# Autodesk Inventor assembly: smartboard1
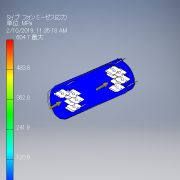
[picture p0: Inventor's stored thumbnail of the model, 180x180]
Saved by Autodesk Inventor 2019 (Build 230136000, 136)
## iProperties
Created: 2019-02-09
Part Number: smartboard1
Material: 一般
Document SubType Name: Assembly
Designer: drago
Author: drago
## Documents named in this file (15)
- C:\Users\drago\Documents\SFP\sfp_smartboard\smartboard1.iam
- C:\Users\drago\Documents\SFP\sfp_smartboard\sfp_smartboard_lower_deck.ipt
- C:\Users\drago\Documents\SFP\sfp_smartboard\track_data\Truck.iam
- C:\Users\drago\Documents\Inventor\Content Center Files\R2019\ja-JP\DIN 7991(2)\DIN 7991 - M5x20.ipt
- C:\Users\drago\Documents\Inventor\Content Center Files\R2019\ja-JP\AS 1112 (2)\AS 1112 - M5  Type 5.ipt
- C:\Users\drago\Documents\SFP\sfp_smartboard\sc601_load_cell.ipt
- C:\Users\drago\Documents\Inventor\Content Center Files\R2019\ja-JP\AS 1112 (2)\AS 1112 - M6  Type 5.ipt
- C:\Users\drago\Documents\Inventor\Content Center Files\R2019\ja-JP\AS 1427(04)\AS 1427 - M6 x 50(5) I.ipt
- C:\Users\drago\Documents\SFP\sfp_smartboard\sfp_smartboard_upper_deck.ipt
- C:\Users\drago\Documents\SFP\sfp_smartboard\smartboard1\AIP\FEA\cs536vov4.fins
- C:\Users\drago\Documents\SFP\sfp_smartboard\smartboard1\AIP\FEA\cs536vow0.fsat
- C:\Users\drago\Documents\SFP\sfp_smartboard\smartboard1\AIP\FEA\cs536vow0.ftes
- C:\Users\drago\Documents\SFP\sfp_smartboard\smartboard1\AIP\FEA\cs536vow0.fwiz
- C:\Users\drago\Documents\SFP\sfp_smartboard\smartboard1\AIP\FEA\cs536vp6o.fmsh
- C:\Users\drago\Documents\SFP\sfp_smartboard\smartboard1\AIP\FEA\cs536vp6p.fres
## Components (54 placed, 8 different names)
1. sfp_smartboard_lower_deck:1 — 挿入:2, 挿入:3, 挿入:4, 挿入:5, 挿入:6, 挿入:7, 挿入:8, 挿入:9, 挿入:10, 挿入:11, 挿入:12, 挿入:13, メイト:1, メイト:2, 挿入:22, 挿入:24, メイト:6, メイト:7, 挿入:27, 挿入:29
2. Truck:1 [sub-assembly] — 挿入:9, 挿入:10, 挿入:18, 挿入:19, 挿入:20, 挿入:21
3. Truck:2 [sub-assembly] — 挿入:11, 挿入:13, 挿入:14, 挿入:15, 挿入:16, 挿入:17
4. DIN 7991 M5x20:1 — 挿入:12
5. DIN 7991 M5x20:3 — 挿入:3
6. DIN 7991 M5x20:4 — 挿入:2
7. DIN 7991 M5x20:5 — 挿入:4
8. DIN 7991 M5x20:6 — 挿入:7
9. DIN 7991 M5x20:7 — 挿入:8
10. DIN 7991 M5x20:8 — 挿入:6
11. DIN 7991 M5x20:9 — 挿入:5
12. AS 1112 (2) - Metric M5  Type 5:1 — 挿入:14
13. AS 1112 (2) - Metric M5  Type 5:2 — 挿入:15
14. AS 1112 (2) - Metric M5  Type 5:3 — 挿入:16
15. AS 1112 (2) - Metric M5  Type 5:4 — 挿入:17
16. AS 1112 (2) - Metric M5  Type 5:5 — 挿入:18
17. AS 1112 (2) - Metric M5  Type 5:6 — 挿入:19
18. AS 1112 (2) - Metric M5  Type 5:7 — 挿入:20
19. AS 1112 (2) - Metric M5  Type 5:8 — 挿入:21
20. sc601_load_cell:1 — 挿入:31, 挿入:32, 挿入:33, 挿入:34, 挿入:47, 挿入:51, 挿入:52
21. sc601_load_cell:2 — 挿入:26, メイト:3, メイト:4, メイト:5, 挿入:48, 挿入:49, 挿入:50
22. AS 1112 (2) - Metric M6  Type 5:1 — 挿入:43, 挿入:45
23. AS 1112 (2) - Metric M6  Type 5:2 — 挿入:45, 挿入:47
24. AS 1112 (2) - Metric M6  Type 5:3 — 挿入:42, 挿入:48
25. AS 1112 (2) - Metric M6  Type 5:4 — 挿入:24, 挿入:25
26. AS 1112 (2) - Metric M6  Type 5:5 — 挿入:23, 挿入:26
27. AS 1112 (2) - Metric M6  Type 5:6 — 挿入:22, 挿入:23
28. AS 1112 (2) - Metric M6  Type 5:7 — 挿入:41
29. AS 1112 (2) - Metric M6  Type 5:8 — 挿入:25, メイト:3
30. AS 1112 (2) - Metric M6  Type 5:9 — メイト:4
31. AS 1112 (2) - Metric M6  Type 5:10 — 挿入:44, 挿入:46
32. AS 1112 (2) - Metric M6  Type 5:11 — メイト:5
33. AS 1112 (2) - Metric M6  Type 5:12 — 挿入:40, 挿入:42
34. AS 1112 (2) - Metric M6  Type 5:13 — 挿入:39, 挿入:41
35. AS 1112 (2) - Metric M6  Type 5:14 — 挿入:27, 挿入:28
36. AS 1112 (2) - Metric M6  Type 5:15 — 挿入:51
37. AS 1112 (2) - Metric M6  Type 5:16 — 挿入:52
38. AS 1112 (2) - Metric M6  Type 5:17 — 挿入:28, 挿入:32
39. AS 1112 (2) - Metric M6  Type 5:18 — 挿入:29, 挿入:30
40. AS 1112 (2) - Metric M6  Type 5:19 — 挿入:50
41. AS 1112 (2) - Metric M6  Type 5:20 — 挿入:46
42. AS 1112 (2) - Metric M6  Type 5:21 — 挿入:33
43. AS 1112 (2) - Metric M6  Type 5:22 — 挿入:34
44. AS 1112 (2) - Metric M6  Type 5:23 — 挿入:49
45. AS 1112 (2) - Metric M6  Type 5:24 — 挿入:30, 挿入:31
46. AS 1427 H - Metric M6 x 50:1 — メイト:1
47. AS 1427 H - Metric M6 x 50:2 — メイト:2
48. AS 1427 H - Metric M6 x 50:7 — メイト:7
49. AS 1427 H - Metric M6 x 50:8 — メイト:6
50. AS 1427 H - Metric M6 x 50:9 — 挿入:36
51. AS 1427 H - Metric M6 x 50:10 — 挿入:37
52. AS 1427 H - Metric M6 x 50:11 — 挿入:38
53. AS 1427 H - Metric M6 x 50:12 — 挿入:35
54. sfp_smartboard_upper_deck:1 — 挿入:35, 挿入:36, 挿入:37, 挿入:38, 挿入:39, 挿入:40, 挿入:43, 挿入:44
## Relationships (58: Insert 51, Mate 7)
- 挿入:2 [Insert]: sfp_smartboard_lower_deck:1 ↔ DIN 7991 M5x20:4
- 挿入:3 [Insert]: sfp_smartboard_lower_deck:1 ↔ DIN 7991 M5x20:3
- 挿入:4 [Insert]: sfp_smartboard_lower_deck:1 ↔ DIN 7991 M5x20:5
- 挿入:5 [Insert]: sfp_smartboard_lower_deck:1 ↔ DIN 7991 M5x20:9
- 挿入:6 [Insert]: sfp_smartboard_lower_deck:1 ↔ DIN 7991 M5x20:8
- 挿入:7 [Insert]: sfp_smartboard_lower_deck:1 ↔ DIN 7991 M5x20:6
- 挿入:8 [Insert]: sfp_smartboard_lower_deck:1 ↔ DIN 7991 M5x20:7
- 挿入:9 [Insert]: sfp_smartboard_lower_deck:1 ↔ Truck:1
- 挿入:10 [Insert]: sfp_smartboard_lower_deck:1 ↔ Truck:1
- 挿入:11 [Insert]: sfp_smartboard_lower_deck:1 ↔ Truck:2
- 挿入:12 [Insert]: sfp_smartboard_lower_deck:1 ↔ DIN 7991 M5x20:1
- 挿入:13 [Insert]: sfp_smartboard_lower_deck:1 ↔ Truck:2
- 挿入:14 [Insert]: Truck:2 ↔ AS 1112 (2) - Metric M5  Type 5:1
- 挿入:15 [Insert]: Truck:2 ↔ AS 1112 (2) - Metric M5  Type 5:2
- 挿入:16 [Insert]: Truck:2 ↔ AS 1112 (2) - Metric M5  Type 5:3
- 挿入:17 [Insert]: Truck:2 ↔ AS 1112 (2) - Metric M5  Type 5:4
- 挿入:18 [Insert]: Truck:1 ↔ AS 1112 (2) - Metric M5  Type 5:5
- 挿入:19 [Insert]: Truck:1 ↔ AS 1112 (2) - Metric M5  Type 5:6
- 挿入:20 [Insert]: Truck:1 ↔ AS 1112 (2) - Metric M5  Type 5:7
- 挿入:21 [Insert]: Truck:1 ↔ AS 1112 (2) - Metric M5  Type 5:8
- メイト:1 [Mate]: sfp_smartboard_lower_deck:1 ↔ AS 1427 H - Metric M6 x 50:1
- メイト:2 [Mate]: sfp_smartboard_lower_deck:1 ↔ AS 1427 H - Metric M6 x 50:2
- 挿入:22 [Insert]: sfp_smartboard_lower_deck:1 ↔ AS 1112 (2) - Metric M6  Type 5:6
- 挿入:23 [Insert]: AS 1112 (2) - Metric M6  Type 5:5 ↔ AS 1112 (2) - Metric M6  Type 5:6
- 挿入:24 [Insert]: sfp_smartboard_lower_deck:1 ↔ AS 1112 (2) - Metric M6  Type 5:4
- 挿入:25 [Insert]: AS 1112 (2) - Metric M6  Type 5:4 ↔ AS 1112 (2) - Metric M6  Type 5:8
- 挿入:26 [Insert]: sc601_load_cell:2 ↔ AS 1112 (2) - Metric M6  Type 5:5
- メイト:3 [Mate]: sc601_load_cell:2 ↔ AS 1112 (2) - Metric M6  Type 5:8
- メイト:4 [Mate]: sc601_load_cell:2 ↔ AS 1112 (2) - Metric M6  Type 5:9
- メイト:5 [Mate]: sc601_load_cell:2 ↔ AS 1112 (2) - Metric M6  Type 5:11
- メイト:6 [Mate]: sfp_smartboard_lower_deck:1 ↔ AS 1427 H - Metric M6 x 50:8
- メイト:7 [Mate]: sfp_smartboard_lower_deck:1 ↔ AS 1427 H - Metric M6 x 50:7
- 挿入:27 [Insert]: sfp_smartboard_lower_deck:1 ↔ AS 1112 (2) - Metric M6  Type 5:14
- 挿入:28 [Insert]: AS 1112 (2) - Metric M6  Type 5:14 ↔ AS 1112 (2) - Metric M6  Type 5:17
- 挿入:29 [Insert]: sfp_smartboard_lower_deck:1 ↔ AS 1112 (2) - Metric M6  Type 5:18
- 挿入:30 [Insert]: AS 1112 (2) - Metric M6  Type 5:18 ↔ AS 1112 (2) - Metric M6  Type 5:24
- 挿入:31 [Insert]: sc601_load_cell:1 ↔ AS 1112 (2) - Metric M6  Type 5:24
- 挿入:32 [Insert]: sc601_load_cell:1 ↔ AS 1112 (2) - Metric M6  Type 5:17
- 挿入:33 [Insert]: sc601_load_cell:1 ↔ AS 1112 (2) - Metric M6  Type 5:21
- 挿入:34 [Insert]: sc601_load_cell:1 ↔ AS 1112 (2) - Metric M6  Type 5:22
- 挿入:35 [Insert]: AS 1427 H - Metric M6 x 50:12 ↔ sfp_smartboard_upper_deck:1
- 挿入:36 [Insert]: AS 1427 H - Metric M6 x 50:9 ↔ sfp_smartboard_upper_deck:1
- 挿入:37 [Insert]: AS 1427 H - Metric M6 x 50:10 ↔ sfp_smartboard_upper_deck:1
- 挿入:38 [Insert]: AS 1427 H - Metric M6 x 50:11 ↔ sfp_smartboard_upper_deck:1
- 挿入:39 [Insert]: AS 1112 (2) - Metric M6  Type 5:13 ↔ sfp_smartboard_upper_deck:1
- 挿入:40 [Insert]: AS 1112 (2) - Metric M6  Type 5:12 ↔ sfp_smartboard_upper_deck:1
- 挿入:41 [Insert]: AS 1112 (2) - Metric M6  Type 5:7 ↔ AS 1112 (2) - Metric M6  Type 5:13
- 挿入:42 [Insert]: AS 1112 (2) - Metric M6  Type 5:3 ↔ AS 1112 (2) - Metric M6  Type 5:12
- 挿入:43 [Insert]: AS 1112 (2) - Metric M6  Type 5:1 ↔ sfp_smartboard_upper_deck:1
- 挿入:44 [Insert]: AS 1112 (2) - Metric M6  Type 5:10 ↔ sfp_smartboard_upper_deck:1
- 挿入:45 [Insert]: AS 1112 (2) - Metric M6  Type 5:1 ↔ AS 1112 (2) - Metric M6  Type 5:2
- 挿入:46 [Insert]: AS 1112 (2) - Metric M6  Type 5:10 ↔ AS 1112 (2) - Metric M6  Type 5:20
- 挿入:47 [Insert]: sc601_load_cell:1 ↔ AS 1112 (2) - Metric M6  Type 5:2
- 挿入:48 [Insert]: sc601_load_cell:2 ↔ AS 1112 (2) - Metric M6  Type 5:3
- 挿入:49 [Insert]: sc601_load_cell:2 ↔ AS 1112 (2) - Metric M6  Type 5:23
- 挿入:50 [Insert]: sc601_load_cell:2 ↔ AS 1112 (2) - Metric M6  Type 5:19
- 挿入:51 [Insert]: sc601_load_cell:1 ↔ AS 1112 (2) - Metric M6  Type 5:15
- 挿入:52 [Insert]: sc601_load_cell:1 ↔ AS 1112 (2) - Metric M6  Type 5:16
## Named parameters: sa_0 = 30000, sa_1 = 200 mm, sa_2 = -25 mm, sa_3 = 0 mm, sa_4 = 30000, sa_5 = 600 mm, sa_6 = -25 mm, sa_7 = 340 mm
note: some values were not read from the file. Shown as the stored number, unit unknown: "sa_0", "sa_4".
